# Autodesk Inventor assembly: canaleta3
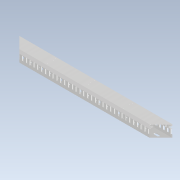
[picture p0: Inventor's stored thumbnail of the model, 180x180]
Saved by Autodesk Inventor 2021 (Build 250183000, 183)
## iProperties
Created: 2021-08-23
Part Number: canaleta3
Document SubType Name: Assembly
Designer: Andrés Holguín
Author: Andrés Holguín
## Documents named in this file (2)
- C:\Users\andre\Documents\GitHub\Dis.-Mecatronico-E6\inventor proyecto\Tablero\Canaletas\canaleta3.iam
- C:\Users\andre\Documents\GitHub\Dis.-Mecatronico-E6\inventor proyecto\Tablero\Canaletas\7308-1.iam
## Components (4 placed, 1 different names)
1. 7308-1:1 [sub-assembly]
2. 7308-1:2 [sub-assembly]
3. 7308-1:3 [sub-assembly] — Mate:1, Angle:1
4. 7308-1:4 [sub-assembly] — Mate:2, Angle:2
## Relationships (7: WeldJoint 3, Mate 2, Angle 2)
- [WeldJoint]: 7308-1:1 ↔ 7308-1:2
- [WeldJoint]: 7308-1:1 ↔ 7308-1:3
- [WeldJoint]: 7308-1:2 ↔ 7308-1:4
- Mate:1: 7308-1:3
- Angle:1 (45 deg): 7308-1:3
- Mate:2: 7308-1:4
- Angle:2 (-45 deg): 7308-1:4
